# Autodesk Inventor assembly: Full_Assembly
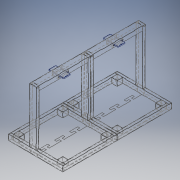
[picture p0: Inventor's stored thumbnail of the model, 180x180]
Saved by Autodesk Inventor 2019 (Build 230136000, 136)
## iProperties
Created: 2018-09-08
Part Number: Full_Assembly
Document SubType Name: Assembly
Designer: William
Author: William
## Documents named in this file (2)
- C:\Users\William\Documents\Simon_PennApps_F18\Full_Assembly.iam
- C:\Users\William\Documents\Simon_PennApps_F18\Playfield_Assembly.iam
## Components (2 placed, 1 different names)
1. Playfield_Assembly:1 [sub-assembly] — Flush:1, Flush:2, Mate:1
2. Playfield_Assembly:2 [sub-assembly] — Flush:1, Flush:2, Mate:1
## Relationships (3: Flush 2, Mate 1)
- Flush:1: Playfield_Assembly:1 ↔ Playfield_Assembly:2
- Flush:2: Playfield_Assembly:1 ↔ Playfield_Assembly:2
- Mate:1: Playfield_Assembly:1 ↔ Playfield_Assembly:2
